# Autodesk Inventor assembly: Assembly FW
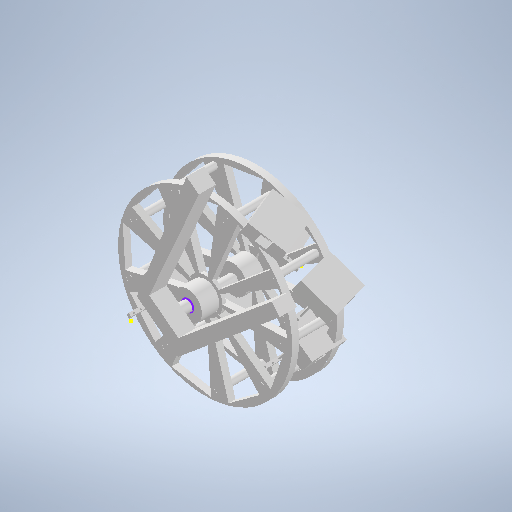
[picture p0: Inventor's stored thumbnail of the model, 512x512]
Saved by Autodesk Inventor 2025.1 (Build 291241000, 241)
## iProperties
Created: 2025-04-19
Part Number: Assembly FW
Document SubType Name: Assembly
Designer: POORNIMA HIREMATH
Author: POORNIMA HIREMATH
## Documents named in this file (7)
- C:\Users\POORNIMA HIREMATH\Documents\Assembly FW.iam
- C:\Users\POORNIMA HIREMATH\Documents\F11.ipt
- C:\Users\POORNIMA HIREMATH\Documents\F22.ipt
- C:\Users\POORNIMA HIREMATH\Documents\F 3.ipt
- C:\Users\POORNIMA HIREMATH\Documents\F4.ipt
- C:\Users\POORNIMA HIREMATH\Documents\F stand.ipt
- C:\Users\POORNIMA HIREMATH\Documents\Assembly3.4.iam
## Components (21 placed, 6 different names)
1. F22:1 — Rotational:4, Rotational:5, Rotational:6, Rotational:7
2. F11:4 — Rotational:5
3. F 3:2 — Rotational:4, Rotational:8, Rotational:9, Rotational:10, Rotational:11, Rotational:12, Rotational:13, Rotational:14, Rotational:15, Rotational:16
4. F 3:3 — Rotational:6, Rotational:17
5. F11:5 — Rotational:7
6. F4:1 — Rotational:8
7. F4:2 — Rotational:9
8. F4:3 — Rotational:10
9. F4:4 — Rotational:11
10. F4:5 — Rotational:12
11. F4:6 — Rotational:16
12. F4:7 — Rotational:15
13. F4:8 — Rotational:14
14. F4:9 — Rotational:13
15. F stand:1 — Rotational:17
16. Assembly3.4:1 [sub-assembly]
17. Assembly3.4:2 [sub-assembly]
18. Assembly3.4:3 [sub-assembly]
19. Assembly3.4:4 [sub-assembly]
20. Assembly3.4:5 [sub-assembly]
21. Assembly3.4:7 [sub-assembly]
## Relationships (14: RevoluteJoint 14)
- Rotational:4 [RevoluteJoint]: F22:1 ↔ F 3:2
- Rotational:5 [RevoluteJoint]: F22:1 ↔ F11:4
- Rotational:6 [RevoluteJoint]: F22:1 ↔ F 3:3
- Rotational:7 [RevoluteJoint]: F22:1 ↔ F11:5
- Rotational:8 [RevoluteJoint]: F 3:2 ↔ F4:1
- Rotational:9 [RevoluteJoint]: F 3:2 ↔ F4:2
- Rotational:10 [RevoluteJoint]: F 3:2 ↔ F4:3
- Rotational:11 [RevoluteJoint]: F 3:2 ↔ F4:4
- Rotational:12 [RevoluteJoint]: F 3:2 ↔ F4:5
- Rotational:13 [RevoluteJoint]: F 3:2 ↔ F4:9
- Rotational:14 [RevoluteJoint]: F 3:2 ↔ F4:8
- Rotational:15 [RevoluteJoint]: F 3:2 ↔ F4:7
- Rotational:16 [RevoluteJoint]: F 3:2 ↔ F4:6
- Rotational:17 [RevoluteJoint]: F 3:3 ↔ F stand:1
